# Autodesk Inventor assembly: Electrical_Component_Arrangment
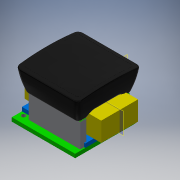
[picture p0: Inventor's stored thumbnail of the model, 180x180]
Saved by Autodesk Inventor 2019.4 (Build 234330000, 330)
## iProperties
Created: 2021-06-29
Part Number: Electrical_Component_Arrangment
Document SubType Name: Assembly
Designer: keshav
Author: keshav
## Documents named in this file (7)
- D:\Keshav\Maker\Microview_Pendant\Microview_Pendant\CAD\Electrical_Component_Arrangment.iam
- D:\Keshav\Maker\Microview_Pendant\Microview_Pendant\CAD\Vero_Board.ipt
- D:\Keshav\Maker\Microview_Pendant\Microview_Pendant\CAD\Wavgat_Battery_Charger.ipt
- D:\Keshav\Micro Controlers\CAD of controllers\sparkfun-microview-oled-1.snapshot.3\Sparkfun display.ipt
- D:\Keshav\Maker\Microview_Pendant\Microview_Pendant\CAD\Female_Header_Spacer.ipt
- D:\Keshav\Maker\Microview_Pendant\Microview_Pendant\CAD\Battery_37v_270mAh.ipt
- D:\Keshav\Maker\Microview_Pendant\Microview_Pendant\CAD\Push_Button.ipt
## Components (7 placed, 6 different names)
1. Vero_Board:1 — Flush:1, Flush:2, Flush:8, Flush:10, Mate:1, Flush:11, Mate:6, Flush:15
2. Wavgat_Battery_Charger:1 — Flush:1, Flush:2, Mate:1, Flush:14
3. Sparkfun display:1 — Flush:12, Flush:13, Mate:4
4. Female_Header_Spacer:1 — Flush:5, Flush:6, Flush:8, Flush:10, Flush:11, Mate:2, Mate:3
5. Female_Header_Spacer:2 — Flush:5, Flush:6, Mate:2, Flush:12, Flush:13, Mate:5
6. Battery_37v_270mAh:1 — Mate:3, Mate:4, Flush:14
7. Push_Button:1 — Mate:5, Mate:6, Flush:15
## Relationships (17: Flush 11, Mate 6)
- Flush:1: Vero_Board:1 ↔ Wavgat_Battery_Charger:1
- Flush:2 (4.2 mm): Vero_Board:1 ↔ Wavgat_Battery_Charger:1
- Flush:5: Female_Header_Spacer:1 ↔ Female_Header_Spacer:2
- Flush:6: Female_Header_Spacer:1 ↔ Female_Header_Spacer:2
- Flush:8 (2.6 mm): Vero_Board:1 ↔ Female_Header_Spacer:1
- Flush:10 (4.4 mm): Vero_Board:1 ↔ Female_Header_Spacer:1
- Mate:1: Vero_Board:1 ↔ Wavgat_Battery_Charger:1
- Flush:11: Vero_Board:1 ↔ Female_Header_Spacer:1
- Mate:2 (15.4 mm): Female_Header_Spacer:1 ↔ Female_Header_Spacer:2
- Flush:12 (1.5 mm): Sparkfun display:1 ↔ Female_Header_Spacer:2
- Flush:13 (1.55 mm): Sparkfun display:1 ↔ Female_Header_Spacer:2
- Mate:3 (0.2 mm): Female_Header_Spacer:1 ↔ Battery_37v_270mAh:1
- Mate:4: Sparkfun display:1 ↔ Battery_37v_270mAh:1
- Flush:14: Wavgat_Battery_Charger:1 ↔ Battery_37v_270mAh:1
- Mate:5 (1.5 mm): Female_Header_Spacer:2 ↔ Push_Button:1
- Mate:6: Vero_Board:1 ↔ Push_Button:1
- Flush:15 (8 mm): Vero_Board:1 ↔ Push_Button:1
